# Autodesk Inventor assembly: ServoHousingAssembly
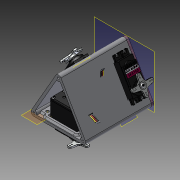
[picture p0: Inventor's stored thumbnail of the model, 180x180]
Saved by Autodesk Inventor 2014 SP1 (Build 180222100, 222)
## iProperties
Created: 2014-11-03
Part Number: ServoHousingAssembly
Document SubType Name: Assembly
Designer: rawrdong
Author: rawrdong
## Documents named in this file (4)
- C:\Users\rawrdong\Documents\GitHub\FlippityFlappity\CAD_HW\ServoHousingAssembly.iam
- C:\Users\rawrdong\Documents\GitHub\FlippityFlappity\CAD_HW\servo-6.snapshot.1\Imported Components\Servo HS425BB\Servo HS425BB.ipt
- C:\Users\rawrdong\Documents\GitHub\FlippityFlappity\CAD_HW\ServoHousingEndPlates.ipt
- C:\Users\rawrdong\Documents\GitHub\FlippityFlappity\CAD_HW\ServoHousingTest.ipt
## Components (5 placed, 3 different names)
1. Servo HS425BB:1 — Mate:3
2. Servo HS425BB:2 — Mate:2
3. Servo HS425BB:3 — Mate:1
4. ServoHousingEndPlates:1 — Mate:4, Mate:5, Mate:6
5. ServoHousingTest:2 — Mate:1, Mate:2, Mate:3, Mate:4, Mate:5, Mate:6
## Relationships (6: Mate 6)
- Mate:1: Servo HS425BB:3 ↔ ServoHousingTest:2
- Mate:2: Servo HS425BB:2 ↔ ServoHousingTest:2
- Mate:3: Servo HS425BB:1 ↔ ServoHousingTest:2
- Mate:4: ServoHousingEndPlates:1 ↔ ServoHousingTest:2
- Mate:5: ServoHousingEndPlates:1 ↔ ServoHousingTest:2
- Mate:6: ServoHousingEndPlates:1 ↔ ServoHousingTest:2
